# Autodesk Inventor assembly: Robot
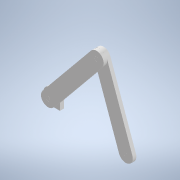
[picture p0: Inventor's stored thumbnail of the model, 180x180]
Saved by Autodesk Inventor 2021 (Build 250183000, 183)
## iProperties
Created: 2022-01-12
Part Number: Robot
Document SubType Name: Assembly
Designer: Yeison
Author: Yeison
## Documents named in this file (4)
- C:\Users\Yeison\Documents\GitHub\Servomecanismos\Modelo 2021\Robot.iam
- C:\Users\Yeison\Documents\GitHub\Servomecanismos\Modelo 2021\Soporte.ipt
- C:\Users\Yeison\Documents\GitHub\Servomecanismos\Modelo 2021\pin2.ipt
- C:\Users\Yeison\Documents\GitHub\Servomecanismos\Modelo 2021\Eslabon.ipt
## Components (6 placed, 3 different names)
1. Soporte:1 — Rigid:1
2. pin2:1 — Rigid:1, Rotational:1
3. Eslabon:1 — Rotational:1, Rotational:2, Rotational:3
4. pin2:2 — Rotational:2
5. Eslabon:2 — Rotational:3, Rigid:2
6. pin2:3 — Rigid:2
## Relationships (5: RevoluteJoint 3, WeldJoint 2)
- Rigid:1 [WeldJoint]: Soporte:1 ↔ pin2:1
- Rotational:1 [RevoluteJoint]: pin2:1 ↔ Eslabon:1
- Rotational:2 [RevoluteJoint]: Eslabon:1 ↔ pin2:2
- Rotational:3 [RevoluteJoint]: Eslabon:1 ↔ Eslabon:2
- Rigid:2 [WeldJoint]: Eslabon:2 ↔ pin2:3
